# Autodesk Inventor assembly: Arm 2.0 Assembly
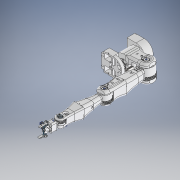
[picture p0: Inventor's stored thumbnail of the model, 180x180]
Saved by Autodesk Inventor 2017 SP1 (Build 210196100, 196)
## iProperties
Created: 2017-09-28
Part Number: Arm 2.0 Assembly
Document SubType Name: Assembly
Designer: Zach
Author: Zach
## Documents named in this file (58)
- C:\Users\Zach\Documents\GitHub\tr1\src\Body\Arm 2.0 Assembly\Arm 2.0 Assembly.iam
- C:\Users\Zach\Documents\GitHub\tr1\src\Body\Arm 2.0 Assembly\Steel Rod 8mm x 135mm.ipt
- C:\Users\Zach\Documents\GitHub\tr1\lib\22x8x8mm Bearing.ipt
- C:\Users\Zach\Documents\GitHub\tr1\src\Body\Arm 2.0 Assembly\AA004.ipt
- C:\Users\Zach\Documents\GitHub\tr1\lib\QS12MM250\QS12MM250.ipt
- C:\Users\Zach\Documents\GitHub\tr1\src\Body\Arm 2.0 Assembly\Steel Rod 8mm x 100mm.ipt
- C:\Users\Zach\Documents\GitHub\tr1\src\Body\Arm 2.0 Assembly\AA013.ipt
- C:\Users\Zach\Documents\GitHub\tr1\src\Body\Arm 2.0 Assembly\AA014.ipt
- C:\Users\Zach\Documents\GitHub\tr1\lib\12V DC Motor 378-1.ipt
- C:\Users\Zach\Documents\Inventor\Content Center Files\R2017\en-US\ISO 4017(1)\ISO 4017 - M5 x 20 - ISO.ipt
- C:\Users\Zach\Documents\GitHub\tr1\src\Body\Arm 2.0 Assembly\Steel Rod 8mm x 80mm.ipt
- C:\Users\Zach\Documents\GitHub\BCN3D-Moveo\Autodesk Inventor files\Gripper B Assembly.iam
- C:\Users\Zach\Documents\Inventor\Content Center Files\R2017\en-US\CNS 4320\CNS 4320 - M8 x 1 x 100.ipt
- C:\Users\Zach\Documents\GitHub\tr1\lib\AS 1110 - M8 x 150.ipt
- C:\Users\Zach\Documents\GitHub\tr1\lib\8mm Hub.ipt
- C:\Users\Zach\Documents\GitHub\tr1\src\Body\Arm 2.0 Assembly\Arm 2.0 Assembly\Design Accelerator\Spur Gears5.iam
- C:\Users\Zach\Documents\GitHub\tr1\lib\4mm mounting hub.ipt
- C:\Users\Zach\Documents\GitHub\tr1\lib\6201RS\6201RS.ipt
- C:\Users\Zach\Documents\GitHub\tr1\lib\U51105\U51105.ipt
- C:\Users\Zach\Documents\GitHub\tr1\src\Body\Arm 2.0 Assembly\AA031.ipt
- C:\Users\Zach\Documents\GitHub\tr1\src\Body\Arm 2.0 Assembly\AA034.ipt
- C:\Users\Zach\Documents\GitHub\tr1\src\Body\Arm 2.0 Assembly\Arm 2.0 Assembly\Design Accelerator\Spur Gears6.iam
- C:\Users\Zach\Documents\GitHub\tr1\src\Body\Arm 2.0 Assembly\AA008c.ipt
- C:\Users\Zach\Documents\GitHub\tr1\src\Body\Arm 2.0 Assembly\AA008d.ipt
- C:\Users\Zach\Documents\GitHub\tr1\src\Body\Arm 2.0 Assembly\AA035.ipt
- C:\Users\Zach\Documents\GitHub\tr1\src\Body\Arm 2.0 Assembly\Arm 2.0 Assembly\Design Accelerator\Spur Gears7.iam
- C:\Users\Zach\Documents\GitHub\tr1\src\Body\Arm 2.0 Assembly\AA036.ipt
- C:\Users\Zach\Documents\GitHub\tr1\src\Body\Arm 2.0 Assembly\AA037.ipt
- C:\Users\Zach\Documents\GitHub\tr1\src\Body\Arm 2.0 Assembly\AA016b.ipt
- C:\Users\Zach\Documents\GitHub\tr1\src\Body\Arm 2.0 Assembly\AA005b.ipt
- C:\Users\Zach\Documents\GitHub\tr1\src\Body\Arm 2.0 Assembly\AA006b.ipt
- C:\Users\Zach\Documents\GitHub\tr1\src\Body\Arm 2.0 Assembly\AA001c.ipt
- C:\Users\Zach\Documents\GitHub\tr1\lib\uxcell 12V 5RPM 8mm Worm Gear Motor\uxcell 12V 5RPM 8mm Worm Gear Motor.ipt
- C:\Users\Zach\Documents\GitHub\tr1\lib\Bourns ACE 128\Bourns ACE 128.ipt
- C:\Users\Zach\Documents\GitHub\tr1\src\Body\Arm 2.0 Assembly\Arm 2.0 Assembly\Design Accelerator\Spur Gears8.iam
- C:\Users\Zach\Documents\GitHub\tr1\src\Body\Arm 2.0 Assembly\Arm 2.0 Assembly\Design Accelerator\Spur Gears11.iam
- C:\Users\Zach\Documents\GitHub\tr1\src\Body\Arm 2.0 Assembly\Arm 2.0 Assembly\Design Accelerator\Spur Gears9.iam
- C:\Users\Zach\Documents\GitHub\tr1\src\Body\Arm 2.0 Assembly\AA010b.ipt
- C:\Users\Zach\Documents\GitHub\tr1\lib\uxcell 12V 6RPM 6mm Worm Gear Motor\uxcell 12V 6RPM 6mm Worm Gear Motor.ipt
- C:\Users\Zach\Documents\GitHub\tr1\src\Body\Arm 2.0 Assembly\Arm 2.0 Assembly\Design Accelerator\Spur Gears10.iam
- C:\Users\Zach\Documents\GitHub\tr1\src\Body\Arm 2.0 Assembly\Arm 2.0 Assembly\Design Accelerator\Spur Gears12.iam
- C:\Users\Zach\Documents\GitHub\tr1\src\Body\Arm 2.0 Assembly\AA041.ipt
- C:\Users\Zach\Documents\GitHub\tr1\src\Body\Arm 2.0 Assembly\AA042.ipt
- C:\Users\Zach\Documents\Inventor\Content Center Files\R2017\en-US\ISO 7045  H\ISO 7045 - M3 x 8 - 4.8 - H - ISO.ipt
- C:\Users\Zach\Documents\GitHub\tr1\src\Body\Arm 2.0 Assembly\AA043.ipt
- C:\Users\Zach\Documents\GitHub\tr1\src\Body\Arm 2.0 Assembly\AA044.ipt
- C:\Users\Zach\Documents\GitHub\tr1\src\Body\Arm 2.0 Assembly\AA045.ipt
- C:\Users\Zach\Documents\GitHub\tr1\src\Body\Arm 2.0 Assembly\Arm 2.0 Assembly\Design Accelerator\Spur Gears13.iam
- C:\Users\Zach\Documents\GitHub\tr1\src\Body\Arm 2.0 Assembly\Arm 2.0 Assembly\Design Accelerator\Spur Gears16.iam
- C:\Users\Zach\Documents\GitHub\tr1\src\Body\Arm 2.0 Assembly\AA046.ipt
- C:\Users\Zach\Documents\GitHub\tr1\lib\MG995.ipt
- C:\Users\Zach\Documents\GitHub\tr1\lib\Servo Mounting Hub.ipt
- C:\Users\Zach\Documents\GitHub\tr1\src\Body\Arm 2.0 Assembly\AA047.ipt
- C:\Users\Zach\Documents\GitHub\tr1\src\Body\Arm 2.0 Assembly\AA048.ipt
- C:\Users\Zach\Documents\Inventor\Content Center Files\R2017\en-US\ISO 4018\ISO 4018 - M5 x 10.ipt
- C:\Users\Zach\Documents\Inventor\Content Center Files\R2017\en-US\ISO 4018\ISO 4018 - M5 x 25.ipt
- C:\Users\Zach\Documents\Inventor\Content Center Files\R2017\en-US\ISO 7045  H\ISO 7045 - M3 x 12 - 4.8 - H - ISO.ipt
- C:\Users\Zach\Documents\GitHub\tr1\src\Body\Arm 2.0 Assembly\AA049.ipt
## Components (115 placed, 48 different names)
1. AA001c:1 — Mate:554, Mate:555, Mate:556, Mate:557, Mate:560, Flush:18, Mate:562, Mate:563, Mate:564, Mate:565, Mate:566, Mate:567, Mate:568, Mate:569, Mate:570, Mate:571, Mate:572, Mate:573, Mate:574, Mate:576, Mate:578, Mate:581, Angle:1, Mate:592, Mate:602
2. AA004:1 — Mate:23, Mate:345, Mate:347, Mate:350, Mate:357, Mate:554, Mate:555, Mate:556, Mate:590, Mate:591
3. AA005b:1 — Mate:537, Mate:538, Mate:539, Mate:541, Mate:542, Mate:543
4. AA006b:1 — Mate:544, Mate:583, Mate:584, Angle:2, Mate:588, Mate:593, Mate:594, Mate:598, Mate:599, Mate:600, Mate:609
5. AA008c:1 — Mate:449, Mate:450, Mate:451, Mate:452, Mate:453, Mate:454, Mate:463, Mate:464, Mate:466, Mate:467, Mate:481, Mate:616, Mate:662, Mate:663, Mate:751
6. AA008d:1 — Mate:455, Mate:456, Mate:457, Mate:461, Mate:463, Mate:464, Mate:466, Mate:467, Mate:614, Angle:4, Mate:635, Mate:662, Mate:663, Mate:697, Mate:699, Mate:751
7. AA010b:1 — Mate:615, Mate:616, Mate:617, Mate:618, Mate:620, Mate:621, Mate:623, Mate:624, Mate:625, Mate:626, Mate:628, Mate:630, Mate:632, Mate:633, Mate:634, Mate:636, Mate:637, Angle:6, Mate:642, Flush:20, Mate:648, Mate:650
8. AA013:2 — Mate:142, Mate:143, Mate:144, Mate:145, Mate:146, Mate:147, Mate:563, Mate:564, Mate:565
9. AA014:2 — Mate:628, Mate:629, Mate:630
10. AA016b:1 — Mate:518, Mate:519, Mate:520, Mate:521, Mate:525, Mate:526, Mate:527, Mate:529, Mate:530, Mate:664, Mate:665, Mate:667, Mate:668, Mate:669, Angle:7, Mate:671, Mate:673, Mate:675, Mate:676, Mate:677
11. AA031:1 — Mate:366, Mate:367, Mate:523, Mate:524
12. AA034:1 — Mate:529, Mate:534, Mate:535, Mate:700, Mate:701, Mate:709
13. AA035:1 — Mate:477, Mate:479, Mate:481, Mate:557, Mate:601, Mate:652, Mate:653, Mate:697, Mate:699
14. AA036:1 — Mate:498, Mate:500, Mate:501, Mate:502, Mate:511, Mate:698
15. AA037:1 — Mate:501, Mate:502, Mate:514, Mate:515, Mate:516, Mate:517, Mate:518, Mate:519, Mate:520, Mate:530, Mate:664, Mate:665, Mate:698
16. AA041:1 — Mate:675, Mate:676, Mate:677, Mate:682, Mate:683, Mate:684, Mate:685
17. AA042:1 — Mate:678, Mate:679, Mate:686, Mate:687, Angle:14
18. AA043:1 — Mate:688, Mate:689, Angle:8
19. AA043:2 — Mate:693, Mate:694, Angle:10
20. AA043:3 — Mate:742, Mate:743, Angle:13
21. AA044:1 — Mate:691, Mate:692, Angle:9
22. AA044:2 — Mate:695, Mate:696, Angle:11
23. AA045:2 — Mate:700, Mate:701, Mate:702, Mate:703, Mate:704, Mate:705, Mate:706, Mate:708, Flush:21, Mate:709, Mate:711, Mate:713, Mate:715, Mate:717, Mate:718, Angle:12, Mate:719, Mate:720, Mate:723, Mate:725, Mate:780, Mate:781, Mate:784, Mate:785
24. AA046:1 — Mate:727, Mate:728, Mate:731, Mate:735, Mate:736, Mate:737, Mate:752, Mate:756, Mate:757, Mate:758, Mate:759, Mate:760, Mate:761, Mate:762, Mate:763
25. AA047:1 — Mate:735, Mate:736, Mate:737, Mate:738, Mate:739, Mate:740, Mate:753, Mate:754, Mate:755, Mate:800, Mate:801
26. AA048:1 — Mate:744, Mate:745, Mate:746, Mate:747, Mate:748, Mate:749
27. AA049:1 — Mate:783, Mate:784, Mate:785, Mate:786, Mate:787, Mate:788, Mate:789, Mate:790, Mate:791
28. Gripper B Assembly:1 [sub-assembly] — Mate:747, Mate:748, Mate:749, Mate:750, Flush:22, Flush:23
29. 22x8x8mm Bearing:1 — Mate:433, Mate:560
30. 22x8x8mm Bearing:2 — Mate:437, Mate:562
31. 22x8x8mm Bearing:3 — Mate:57, Mate:620, Mate:626, Mate:645
32. 22x8x8mm Bearing:4 — Mate:621, Mate:629, Mate:642
33. 22x8x8mm Bearing:5 — Mate:186, Mate:708
34. 22x8x8mm Bearing:6 — Mate:187, Mate:719
35. 22x8x8mm Bearing:7 — Mate:264, Mate:526
36. 22x8x8mm Bearing:8 — Mate:527, Mate:528
37. 22x8x8mm Bearing:13 — Mate:451, Mate:452
38. 22x8x8mm Bearing:14 — Mate:449, Mate:450
39. QS12MM250:1 — Mate:23, Mate:344, Mate:346, Mate:348, Mate:354, Mate:537, Mate:544, Mate:585, Mate:593, Mate:594, Mate:597
40. Steel Rod 8mm x 135mm:1 — Mate:433, Mate:437, Mate:476, Mate:477, Flush:18, Mate:575, Mate:651
41. Steel Rod 8mm x 100mm:1 — Mate:57, Mate:491, Mate:498, Flush:20, Mate:644, Mate:649
42. Steel Rod 8mm x 80mm:1 — Mate:186, Mate:187, Mate:706, Flush:21, Mate:710, Mate:721, Mate:724, Mate:730, Mate:783
43. 12V DC Motor 378-1:3 — Mate:702, Mate:703, Mate:704, Mate:705, Mate:712, Mate:714, Mate:778, Mate:779
44. 12V DC Motor 378-1:4 — Mate:514, Mate:515, Mate:516, Mate:522
45. 12V DC Motor 378-1:6 — Mate:340, Mate:342, Mate:538, Mate:539, Mate:540, Mate:543
46. 12V DC Motor 378-1:7 — Mate:455, Mate:456, Mate:457, Mate:460, Mate:610
47. uxcell 12V 6RPM 6mm Worm Gear Motor:1 — Mate:632, Mate:633, Mate:634
48. uxcell 12V 5RPM 8mm Worm Gear Motor:1 — Mate:568, Mate:569, Mate:570, Mate:571, Mate:572
49. 6201RS:1 — Mate:346, Mate:347
50. 6201RS:2 — Mate:357, Mate:597
51. U51105:1 — Mate:348, Mate:349, Mate:542
52. U51105:2 — Mate:354, Mate:608, Mate:609
53. 8mm Hub:2 — Mate:368, Mate:531, Mate:534, Mate:535
54. 8mm Hub:3 — Mate:617, Mate:618, Mate:690
55. 8mm Hub:4 — Mate:580, Mate:581, Mate:582
56. 8mm Hub:5 — Mate:644, Mate:645, Mate:646
57. 8mm Hub:6 — Mate:651, Mate:652, Mate:653
58. 8mm Hub:7 — Mate:666, Mate:667, Mate:674
59. 8mm Hub:8 — Mate:720, Mate:721, Mate:726
60. 8mm Hub:9 — Mate:727, Mate:728, Mate:730, Mate:756, Mate:764, Mate:765, Mate:766, Mate:767, Mate:768, Mate:769
61. 4mm mounting hub:1 — Mate:340, Mate:343, Mate:540, Mate:541
62. 4mm mounting hub:3 — Mate:366, Mate:367, Mate:517, Mate:522, Mate:523, Mate:524
63. 4mm mounting hub:5 — Mate:513, Mate:622, Mate:623
64. 4mm mounting hub:7 — Mate:460, Mate:461, Mate:611, Mate:613
65. 4mm mounting hub:8 — Mate:714, Mate:715, Mate:716, Mate:782
66. Servo Mounting Hub:1 — Mate:733, Mate:734, Mate:738, Mate:739, Mate:740, Mate:792, Mate:793, Mate:794, Mate:795, Mate:796, Mate:797, Mate:798, Mate:799
67. ISO 4017 M5 x 20:1 — Mate:146, Mate:147
68. ISO 4017 M5 x 20:2 — Mate:144, Mate:145
69. ISO 4017 M5 x 20:3 — Mate:142, Mate:143
70. CNS 4320 M8 x 100:1 — Mate:264, Mate:368, Mate:521, Mate:525, Mate:528, Mate:531, Mate:666, Mate:670
71. AS 1110 - Metric M8 x 80:2 — Mate:453, Mate:454, Angle:5, Mate:615, Mate:690
72. ISO 7045 H M3 x 8 - 4.8 - H:1 — Mate:680, Mate:681
73. ISO 7045 H M3 x 8 - 4.8 - H:2 — Mate:682, Mate:685
74. ISO 7045 H M3 x 8 - 4.8 - H:3 — Mate:683, Mate:684
75. ISO 7045 H M3 x 8 - 4.8 - H:4 — Mate:686, Mate:687
76. Bourns ACE 128:1 — Mate:573, Mate:574, Mate:577, Angle:1, Mate:693, Mate:694
77. Bourns ACE 128:2 — Mate:583, Mate:584, Angle:2, Mate:587, Mate:695, Mate:696
78. Bourns ACE 128:3 — Mate:612, Mate:614, Angle:4, Mate:635, Mate:691, Mate:692
79. Bourns ACE 128:4 — Mate:636, Mate:637, Angle:6, Mate:647, Mate:688, Mate:689
80. Bourns ACE 128:5 — Mate:668, Mate:669, Angle:7, Mate:672, Mate:678, Mate:679
81. Bourns ACE 128:6 — Mate:717, Mate:718, Angle:12, Mate:722, Mate:742, Mate:743
82. Spur Gears:5 [sub-assembly] — Mate:342, Mate:343, Mate:344, Mate:345, Mate:349, Mate:350
83. Spur Gears:6 [sub-assembly] — Mate:476, Mate:479, Mate:566, Mate:567, Mate:601, Mate:602
84. Spur Gears:7 [sub-assembly] — Mate:491, Mate:500, Mate:511, Mate:513, Mate:622, Mate:624, Mate:625
85. Spur Gears:8 [sub-assembly] — Mate:575, Mate:576, Mate:577, Mate:578, Mate:580, Mate:582, Angle:10
86. Spur Gears:9 [sub-assembly] — Mate:585, Mate:587, Mate:588, Mate:590, Mate:591, Mate:592, Mate:608, Angle:11
87. Spur Gears:10 [sub-assembly] — Mate:610, Mate:611, Mate:612, Mate:613, Angle:5, Angle:9
88. Spur Gears:11 [sub-assembly] — Mate:646, Mate:647, Mate:648, Mate:649, Mate:650, Angle:8
89. Spur Gears:12 [sub-assembly] — Mate:670, Mate:671, Mate:672, Mate:673, Mate:674, Mate:680, Mate:681, Angle:14
90. Spur Gears:13 [sub-assembly] — Mate:710, Mate:711, Mate:712, Mate:713, Mate:716, Mate:731, Mate:757, Mate:770, Mate:771, Mate:772, Mate:773, Mate:774, Mate:775, Mate:776, Mate:777, Mate:782
91. Spur Gears:14 [sub-assembly] — Mate:722, Mate:723, Mate:724, Mate:725, Mate:726, Angle:13
92. MG995:1 — Mate:733, Mate:734, Mate:744, Mate:745, Mate:746
93. MG995:2 — Mate:750, Flush:22, Flush:23
94. ISO 4018 M5 x 10:1 — Mate:754, Mate:755
95. ISO 4018 M5 x 10:2 — Mate:752, Mate:753
96. ISO 4018 M5 x 25:2 — Mate:758, Mate:761
97. ISO 4018 M5 x 25:5 — Mate:759, Mate:763
98. ISO 4018 M5 x 25:6 — Mate:760, Mate:762
99. ISO 7045 H M3 x 12 - 4.8 - H:1 — Mate:765, Mate:767
100. ISO 7045 H M3 x 12 - 4.8 - H:3 — Mate:764, Mate:769
101. ISO 7045 H M3 x 12 - 4.8 - H:2 — Mate:766, Mate:768
102. ISO 7045 H M3 x 12 - 4.8 - H:4 — Mate:770, Mate:775
103. ISO 7045 H M3 x 12 - 4.8 - H:5 — Mate:771, Mate:774
104. ISO 7045 H M3 x 12 - 4.8 - H:6 — Mate:773, Mate:777
105. ISO 7045 H M3 x 12 - 4.8 - H:7 — Mate:772, Mate:776
106. ISO 7045 H M3 x 8 - 4.8 - H:5 — Mate:778, Mate:780
107. ISO 7045 H M3 x 8 - 4.8 - H:6 — Mate:779, Mate:781
108. ISO 4018 M5 x 10:5 — Mate:786, Mate:789
109. ISO 4018 M5 x 10:3 — Mate:787, Mate:790
110. ISO 4018 M5 x 10:4 — Mate:788, Mate:791
111. ISO 7045 H M3 x 8 - 4.8 - H:7 — Mate:795, Mate:799
112. ISO 7045 H M3 x 8 - 4.8 - H:8 — Mate:794, Mate:798
113. ISO 7045 H M3 x 8 - 4.8 - H:9 — Mate:792, Mate:796
114. ISO 7045 H M3 x 8 - 4.8 - H:10 — Mate:793, Mate:797
115. ISO 7045 H M3 x 8 - 4.8 - H:11 — Mate:800, Mate:801
## Relationships (315: Mate 297, Angle 13, Flush 5)
- Mate:23: AA004:1 ↔ QS12MM250:1
- Mate:57: 22x8x8mm Bearing:3 ↔ Steel Rod 8mm x 100mm:1
- Mate:142: AA013:2 ↔ ISO 4017 M5 x 20:3
- Mate:143: AA013:2 ↔ ISO 4017 M5 x 20:3
- Mate:144: AA013:2 ↔ ISO 4017 M5 x 20:2
- Mate:145: AA013:2 ↔ ISO 4017 M5 x 20:2
- Mate:146: AA013:2 ↔ ISO 4017 M5 x 20:1
- Mate:147: AA013:2 ↔ ISO 4017 M5 x 20:1
- Mate:186: 22x8x8mm Bearing:5 ↔ Steel Rod 8mm x 80mm:1
- Mate:187: 22x8x8mm Bearing:6 ↔ Steel Rod 8mm x 80mm:1
- Mate:264: 22x8x8mm Bearing:7 ↔ CNS 4320 M8 x 100:1
- Mate:340: 12V DC Motor 378-1:6 ↔ 4mm mounting hub:1
- Mate:342: 12V DC Motor 378-1:6 ↔ Spur Gears:5
- Mate:343: 4mm mounting hub:1 ↔ Spur Gears:5
- Mate:344: QS12MM250:1 ↔ Spur Gears:5
- Mate:345: AA004:1 ↔ Spur Gears:5
- Mate:346: QS12MM250:1 ↔ 6201RS:1
- Mate:347: AA004:1 ↔ 6201RS:1
- Mate:348: QS12MM250:1 ↔ U51105:1
- Mate:349: U51105:1 ↔ Spur Gears:5
- Mate:350: AA004:1 ↔ Spur Gears:5
- Mate:354: QS12MM250:1 ↔ U51105:2
- Mate:357: AA004:1 ↔ 6201RS:2
- Mate:366: AA031:1 ↔ 4mm mounting hub:3
- Mate:367: AA031:1 ↔ 4mm mounting hub:3
- Mate:368: 8mm Hub:2 ↔ CNS 4320 M8 x 100:1
- Mate:433: 22x8x8mm Bearing:1 ↔ Steel Rod 8mm x 135mm:1
- Mate:437: 22x8x8mm Bearing:2 ↔ Steel Rod 8mm x 135mm:1
- Mate:449: AA008c:1 ↔ 22x8x8mm Bearing:14
- Mate:450: AA008c:1 ↔ 22x8x8mm Bearing:14
- Mate:451: AA008c:1 ↔ 22x8x8mm Bearing:13
- Mate:452: AA008c:1 ↔ 22x8x8mm Bearing:13
- Mate:453: AA008c:1 ↔ AS 1110 - Metric M8 x 80:2
- Mate:454: AA008c:1 ↔ AS 1110 - Metric M8 x 80:2
- Mate:455: AA008d:1 ↔ 12V DC Motor 378-1:7
- Mate:456: AA008d:1 ↔ 12V DC Motor 378-1:7
- Mate:457: AA008d:1 ↔ 12V DC Motor 378-1:7
- Mate:460: 12V DC Motor 378-1:7 ↔ 4mm mounting hub:7
- Mate:461: AA008d:1 ↔ 4mm mounting hub:7
- Mate:463: AA008c:1 ↔ AA008d:1
- Mate:464: AA008c:1 ↔ AA008d:1
- Mate:466: AA008c:1 ↔ AA008d:1
- Mate:467: AA008c:1 ↔ AA008d:1
- Mate:476: Steel Rod 8mm x 135mm:1 ↔ Spur Gears:6
- Mate:477: AA035:1 ↔ Steel Rod 8mm x 135mm:1
- Mate:479: AA035:1 ↔ Spur Gears:6
- Mate:481: AA008c:1 ↔ AA035:1
- Mate:491: Steel Rod 8mm x 100mm:1 ↔ Spur Gears:7
- Mate:498: AA036:1 ↔ Steel Rod 8mm x 100mm:1
- Mate:500: AA036:1 ↔ Spur Gears:7
- Mate:501: AA036:1 ↔ AA037:1
- Mate:502: AA036:1 ↔ AA037:1
- Mate:511: AA036:1 ↔ Spur Gears:7
- Mate:513: 4mm mounting hub:5 ↔ Spur Gears:7
- Mate:514: AA037:1 ↔ 12V DC Motor 378-1:4
- Mate:515: AA037:1 ↔ 12V DC Motor 378-1:4
- Mate:516: AA037:1 ↔ 12V DC Motor 378-1:4
- Mate:517: AA037:1 ↔ 4mm mounting hub:3
- Mate:518: AA016b:1 ↔ AA037:1
- Mate:519: AA016b:1 ↔ AA037:1
- Mate:520: AA016b:1 ↔ AA037:1
- Mate:521: AA016b:1 ↔ CNS 4320 M8 x 100:1
- Mate:522: 12V DC Motor 378-1:4 ↔ 4mm mounting hub:3
- Mate:523: AA031:1 ↔ 4mm mounting hub:3
- Mate:524: AA031:1 ↔ 4mm mounting hub:3
- Mate:525: AA016b:1 ↔ CNS 4320 M8 x 100:1
- Mate:526 (0.5 mm): AA016b:1 ↔ 22x8x8mm Bearing:7
- Mate:527 (0.5 mm): AA016b:1 ↔ 22x8x8mm Bearing:8
- Mate:528: 22x8x8mm Bearing:8 ↔ CNS 4320 M8 x 100:1
- Mate:529: AA016b:1 ↔ AA034:1
- Mate:530: AA016b:1 ↔ AA037:1
- Mate:531: 8mm Hub:2 ↔ CNS 4320 M8 x 100:1
- Mate:534: AA034:1 ↔ 8mm Hub:2
- Mate:535: AA034:1 ↔ 8mm Hub:2
- Mate:537: AA005b:1 ↔ QS12MM250:1
- Mate:538: AA005b:1 ↔ 12V DC Motor 378-1:6
- Mate:539: AA005b:1 ↔ 12V DC Motor 378-1:6
- Mate:540: 12V DC Motor 378-1:6 ↔ 4mm mounting hub:1
- Mate:541: AA005b:1 ↔ 4mm mounting hub:1
- Mate:542: AA005b:1 ↔ U51105:1
- Mate:543: AA005b:1 ↔ 12V DC Motor 378-1:6
- Mate:544: AA006b:1 ↔ QS12MM250:1
- Mate:554: AA001c:1 ↔ AA004:1
- Mate:555: AA001c:1 ↔ AA004:1
- Mate:556: AA001c:1 ↔ AA004:1
- Mate:557: AA001c:1 ↔ AA035:1
- Mate:560: AA001c:1 ↔ 22x8x8mm Bearing:1
- Flush:18: AA001c:1 ↔ Steel Rod 8mm x 135mm:1
- Mate:562: AA001c:1 ↔ 22x8x8mm Bearing:2
- Mate:563: AA001c:1 ↔ AA013:2
- Mate:564: AA001c:1 ↔ AA013:2
- Mate:565: AA001c:1 ↔ AA013:2
- Mate:566: AA001c:1 ↔ Spur Gears:6
- Mate:567 (1 mm): AA001c:1 ↔ Spur Gears:6
- Mate:568: AA001c:1 ↔ uxcell 12V 5RPM 8mm Worm Gear Motor:1
- Mate:569: AA001c:1 ↔ uxcell 12V 5RPM 8mm Worm Gear Motor:1
- Mate:570: AA001c:1 ↔ uxcell 12V 5RPM 8mm Worm Gear Motor:1
- Mate:571: AA001c:1 ↔ uxcell 12V 5RPM 8mm Worm Gear Motor:1
- Mate:572: AA001c:1 ↔ uxcell 12V 5RPM 8mm Worm Gear Motor:1
- Mate:573: AA001c:1 ↔ Bourns ACE 128:1
- Mate:574: AA001c:1 ↔ Bourns ACE 128:1
- Mate:575: Steel Rod 8mm x 135mm:1 ↔ Spur Gears:8
- Mate:576: AA001c:1 ↔ Spur Gears:8
- Mate:577: Bourns ACE 128:1 ↔ Spur Gears:8
- Mate:578: AA001c:1 ↔ Spur Gears:8
- Mate:580: 8mm Hub:4 ↔ Spur Gears:8
- Mate:581: AA001c:1 ↔ 8mm Hub:4
- Mate:582: 8mm Hub:4 ↔ Spur Gears:8
- Angle:1 (0 deg): AA001c:1 ↔ Bourns ACE 128:1
- Mate:583: AA006b:1 ↔ Bourns ACE 128:2
- Mate:584: AA006b:1 ↔ Bourns ACE 128:2
- Angle:2 (0 deg): AA006b:1 ↔ Bourns ACE 128:2
- Mate:585: QS12MM250:1 ↔ Spur Gears:9
- Mate:587: Bourns ACE 128:2 ↔ Spur Gears:9
- Mate:588: AA006b:1 ↔ Spur Gears:9
- Mate:590: AA004:1 ↔ Spur Gears:9
- Mate:591: AA004:1 ↔ Spur Gears:9
- Mate:592: AA001c:1 ↔ Spur Gears:9
- Mate:593: AA006b:1 ↔ QS12MM250:1
- Mate:594: AA006b:1 ↔ QS12MM250:1
- Mate:597: QS12MM250:1 ↔ 6201RS:2
- Mate:598: AA006b:1
- Mate:599: AA006b:1
- Mate:600: AA006b:1
- Mate:601: AA035:1 ↔ Spur Gears:6
- Mate:602 (2.5 mm): AA001c:1 ↔ Spur Gears:6
- Mate:608: U51105:2 ↔ Spur Gears:9
- Mate:609: AA006b:1 ↔ U51105:2
- Mate:610: 12V DC Motor 378-1:7 ↔ Spur Gears:10
- Mate:611: 4mm mounting hub:7 ↔ Spur Gears:10
- Mate:612: Bourns ACE 128:3 ↔ Spur Gears:10
- Mate:613: 4mm mounting hub:7 ↔ Spur Gears:10
- Mate:614: AA008d:1 ↔ Bourns ACE 128:3
- Angle:4 (0 deg): AA008d:1 ↔ Bourns ACE 128:3
- Angle:5 (0 deg): AS 1110 - Metric M8 x 80:2 ↔ Spur Gears:10
- Mate:615: AA010b:1 ↔ AS 1110 - Metric M8 x 80:2
- Mate:616: AA008c:1 ↔ AA010b:1
- Mate:617: AA010b:1 ↔ 8mm Hub:3
- Mate:618: AA010b:1 ↔ 8mm Hub:3
- Mate:620: AA010b:1 ↔ 22x8x8mm Bearing:3
- Mate:621: AA010b:1 ↔ 22x8x8mm Bearing:4
- Mate:622: 4mm mounting hub:5 ↔ Spur Gears:7
- Mate:623: AA010b:1 ↔ 4mm mounting hub:5
- Mate:624: AA010b:1 ↔ Spur Gears:7
- Mate:625: AA010b:1 ↔ Spur Gears:7
- Flush:20 (0.5 mm): AA010b:1 ↔ Steel Rod 8mm x 100mm:1
- Mate:626: AA010b:1 ↔ 22x8x8mm Bearing:3
- Mate:628: AA010b:1 ↔ AA014:2
- Mate:629: AA014:2 ↔ 22x8x8mm Bearing:4
- Mate:630: AA010b:1 ↔ AA014:2
- Mate:632: AA010b:1 ↔ uxcell 12V 6RPM 6mm Worm Gear Motor:1
- Mate:633: AA010b:1 ↔ uxcell 12V 6RPM 6mm Worm Gear Motor:1
- Mate:634: AA010b:1 ↔ uxcell 12V 6RPM 6mm Worm Gear Motor:1
- Mate:635: AA008d:1 ↔ Bourns ACE 128:3
- Mate:636: AA010b:1 ↔ Bourns ACE 128:4
- Mate:637: AA010b:1 ↔ Bourns ACE 128:4
- Angle:6 (0 deg): AA010b:1 ↔ Bourns ACE 128:4
- Mate:642: AA010b:1 ↔ 22x8x8mm Bearing:4
- Mate:644: Steel Rod 8mm x 100mm:1 ↔ 8mm Hub:5
- Mate:645: 22x8x8mm Bearing:3 ↔ 8mm Hub:5
- Mate:646: 8mm Hub:5 ↔ Spur Gears:11
- Mate:647: Bourns ACE 128:4 ↔ Spur Gears:11
- Mate:648: AA010b:1 ↔ Spur Gears:11
- Mate:649: Steel Rod 8mm x 100mm:1 ↔ Spur Gears:11
- Mate:650: AA010b:1 ↔ Spur Gears:11
- Mate:651: Steel Rod 8mm x 135mm:1 ↔ 8mm Hub:6
- Mate:652: AA035:1 ↔ 8mm Hub:6
- Mate:653: AA035:1 ↔ 8mm Hub:6
- Mate:662: AA008c:1 ↔ AA008d:1
- Mate:663: AA008c:1 ↔ AA008d:1
- Mate:664: AA016b:1 ↔ AA037:1
- Mate:665: AA016b:1 ↔ AA037:1
- Mate:666: 8mm Hub:7 ↔ CNS 4320 M8 x 100:1
- Mate:667: AA016b:1 ↔ 8mm Hub:7
- Mate:668: AA016b:1 ↔ Bourns ACE 128:5
- Mate:669: AA016b:1 ↔ Bourns ACE 128:5
- Angle:7 (0 deg): AA016b:1 ↔ Bourns ACE 128:5
- Mate:670: CNS 4320 M8 x 100:1 ↔ Spur Gears:12
- Mate:671: AA016b:1 ↔ Spur Gears:12
- Mate:672: Bourns ACE 128:5 ↔ Spur Gears:12
- Mate:673: AA016b:1 ↔ Spur Gears:12
- Mate:674: 8mm Hub:7 ↔ Spur Gears:12
- Mate:675: AA016b:1 ↔ AA041:1
- Mate:676: AA016b:1 ↔ AA041:1
- Mate:677: AA016b:1 ↔ AA041:1
- Mate:678: AA042:1 ↔ Bourns ACE 128:5
- Mate:679: AA042:1 ↔ Bourns ACE 128:5
- Mate:680: ISO 7045 H M3 x 8 - 4.8 - H:1 ↔ Spur Gears:12
- Mate:681: ISO 7045 H M3 x 8 - 4.8 - H:1 ↔ Spur Gears:12
- Mate:682: AA041:1 ↔ ISO 7045 H M3 x 8 - 4.8 - H:2
- Mate:683: AA041:1 ↔ ISO 7045 H M3 x 8 - 4.8 - H:3
- Mate:684: AA041:1 ↔ ISO 7045 H M3 x 8 - 4.8 - H:3
- Mate:685: AA041:1 ↔ ISO 7045 H M3 x 8 - 4.8 - H:2
- Mate:686: AA042:1 ↔ ISO 7045 H M3 x 8 - 4.8 - H:4
- Mate:687: AA042:1 ↔ ISO 7045 H M3 x 8 - 4.8 - H:4
- Mate:688: AA043:1 ↔ Bourns ACE 128:4
- Mate:689: AA043:1 ↔ Bourns ACE 128:4
- Angle:8 (0 deg): AA043:1 ↔ Spur Gears:11
- Mate:690: 8mm Hub:3 ↔ AS 1110 - Metric M8 x 80:2
- Mate:691: AA044:1 ↔ Bourns ACE 128:3
- Mate:692: AA044:1 ↔ Bourns ACE 128:3
- Angle:9 (0 deg): AA044:1 ↔ Spur Gears:10
- Mate:693: AA043:2 ↔ Bourns ACE 128:1
- Mate:694: AA043:2 ↔ Bourns ACE 128:1
- Angle:10 (0 deg): AA043:2 ↔ Spur Gears:8
- Mate:695: AA044:2 ↔ Bourns ACE 128:2
- Mate:696: AA044:2 ↔ Bourns ACE 128:2
- Angle:11 (0 deg): AA044:2 ↔ Spur Gears:9
- Mate:697: AA008d:1 ↔ AA035:1
- Mate:698: AA036:1 ↔ AA037:1
- Mate:699: AA008d:1 ↔ AA035:1
- Mate:700: AA034:1 ↔ AA045:2
- Mate:701: AA034:1 ↔ AA045:2
- Mate:702: AA045:2 ↔ 12V DC Motor 378-1:3
- Mate:703: AA045:2 ↔ 12V DC Motor 378-1:3
- Mate:704: AA045:2 ↔ 12V DC Motor 378-1:3
- Mate:705: AA045:2 ↔ 12V DC Motor 378-1:3
- Mate:706: AA045:2 ↔ Steel Rod 8mm x 80mm:1
- Mate:708: AA045:2 ↔ 22x8x8mm Bearing:5
- Flush:21: AA045:2 ↔ Steel Rod 8mm x 80mm:1
- Mate:709: AA034:1 ↔ AA045:2
- Mate:710: Steel Rod 8mm x 80mm:1 ↔ Spur Gears:13
- Mate:711: AA045:2 ↔ Spur Gears:13
- Mate:712: 12V DC Motor 378-1:3 ↔ Spur Gears:13
- Mate:713: AA045:2 ↔ Spur Gears:13
- Mate:714: 12V DC Motor 378-1:3 ↔ 4mm mounting hub:8
- Mate:715: AA045:2 ↔ 4mm mounting hub:8
- Mate:716: 4mm mounting hub:8 ↔ Spur Gears:13
- Mate:717: AA045:2 ↔ Bourns ACE 128:6
- Mate:718: AA045:2 ↔ Bourns ACE 128:6
- Angle:12 (0 deg): AA045:2 ↔ Bourns ACE 128:6
- Mate:719: AA045:2 ↔ 22x8x8mm Bearing:6
- Mate:720: AA045:2 ↔ 8mm Hub:8
- Mate:721: Steel Rod 8mm x 80mm:1 ↔ 8mm Hub:8
- Mate:722: Bourns ACE 128:6 ↔ Spur Gears:14
- Mate:723: AA045:2 ↔ Spur Gears:14
- Mate:724: Steel Rod 8mm x 80mm:1 ↔ Spur Gears:14
- Mate:725: AA045:2 ↔ Spur Gears:14
- Mate:726: 8mm Hub:8 ↔ Spur Gears:14
- Mate:727: AA046:1 ↔ 8mm Hub:9
- Mate:728: AA046:1 ↔ 8mm Hub:9
- Mate:730: Steel Rod 8mm x 80mm:1 ↔ 8mm Hub:9
- Mate:731: AA046:1 ↔ Spur Gears:13
- Mate:733: Servo Mounting Hub:1 ↔ MG995:1
- Mate:734: Servo Mounting Hub:1 ↔ MG995:1
- Mate:735: AA046:1 ↔ AA047:1
- Mate:736: AA046:1 ↔ AA047:1
- Mate:737: AA046:1 ↔ AA047:1
- Mate:738: AA047:1 ↔ Servo Mounting Hub:1
- Mate:739: AA047:1 ↔ Servo Mounting Hub:1
- Mate:740: AA047:1 ↔ Servo Mounting Hub:1
- Mate:742: AA043:3 ↔ Bourns ACE 128:6
- Mate:743: AA043:3 ↔ Bourns ACE 128:6
- Angle:13 (0 deg): AA043:3 ↔ Spur Gears:14
- Mate:744: AA048:1 ↔ MG995:1
- Mate:745 (0.5 mm): AA048:1 ↔ MG995:1
- Mate:746 (0.5 mm): AA048:1 ↔ MG995:1
- Mate:747: AA048:1 ↔ Gripper B Assembly:1
- Mate:748: AA048:1 ↔ Gripper B Assembly:1
- Mate:749: AA048:1 ↔ Gripper B Assembly:1
- Mate:750: Gripper B Assembly:1 ↔ MG995:2
- Flush:22 (-2 mm): Gripper B Assembly:1 ↔ MG995:2
- Flush:23 (-0.5 mm): Gripper B Assembly:1 ↔ MG995:2
- Angle:14 (0 deg): AA042:1 ↔ Spur Gears:12
- Mate:751: AA008c:1 ↔ AA008d:1
- Mate:752: AA046:1 ↔ ISO 4018 M5 x 10:2
- Mate:753: AA047:1 ↔ ISO 4018 M5 x 10:2
- Mate:754: AA047:1 ↔ ISO 4018 M5 x 10:1
- Mate:755: AA047:1 ↔ ISO 4018 M5 x 10:1
- Mate:756: AA046:1 ↔ 8mm Hub:9
- Mate:757: AA046:1 ↔ Spur Gears:13
- Mate:758: AA046:1 ↔ ISO 4018 M5 x 25:2
- Mate:759: AA046:1 ↔ ISO 4018 M5 x 25:5
- Mate:760: AA046:1 ↔ ISO 4018 M5 x 25:6
- Mate:761: AA046:1 ↔ ISO 4018 M5 x 25:2
- Mate:762: AA046:1 ↔ ISO 4018 M5 x 25:6
- Mate:763: AA046:1 ↔ ISO 4018 M5 x 25:5
- Mate:764: 8mm Hub:9 ↔ ISO 7045 H M3 x 12 - 4.8 - H:3
- Mate:765: 8mm Hub:9 ↔ ISO 7045 H M3 x 12 - 4.8 - H:1
- Mate:766: 8mm Hub:9 ↔ ISO 7045 H M3 x 12 - 4.8 - H:2
- Mate:767: 8mm Hub:9 ↔ ISO 7045 H M3 x 12 - 4.8 - H:1
- Mate:768: 8mm Hub:9 ↔ ISO 7045 H M3 x 12 - 4.8 - H:2
- Mate:769: 8mm Hub:9 ↔ ISO 7045 H M3 x 12 - 4.8 - H:3
- Mate:770: Spur Gears:13 ↔ ISO 7045 H M3 x 12 - 4.8 - H:4
- Mate:771: Spur Gears:13 ↔ ISO 7045 H M3 x 12 - 4.8 - H:5
- Mate:772: Spur Gears:13 ↔ ISO 7045 H M3 x 12 - 4.8 - H:7
- Mate:773: Spur Gears:13 ↔ ISO 7045 H M3 x 12 - 4.8 - H:6
- Mate:774: Spur Gears:13 ↔ ISO 7045 H M3 x 12 - 4.8 - H:5
- Mate:775: Spur Gears:13 ↔ ISO 7045 H M3 x 12 - 4.8 - H:4
- Mate:776: Spur Gears:13 ↔ ISO 7045 H M3 x 12 - 4.8 - H:7
- Mate:777: Spur Gears:13 ↔ ISO 7045 H M3 x 12 - 4.8 - H:6
- Mate:778: 12V DC Motor 378-1:3 ↔ ISO 7045 H M3 x 8 - 4.8 - H:5
- Mate:779: 12V DC Motor 378-1:3 ↔ ISO 7045 H M3 x 8 - 4.8 - H:6
- Mate:780: AA045:2 ↔ ISO 7045 H M3 x 8 - 4.8 - H:5
- Mate:781: AA045:2 ↔ ISO 7045 H M3 x 8 - 4.8 - H:6
- Mate:782: 4mm mounting hub:8 ↔ Spur Gears:13
- Mate:783: AA049:1 ↔ Steel Rod 8mm x 80mm:1
- Mate:784: AA045:2 ↔ AA049:1
- Mate:785: AA045:2 ↔ AA049:1
- Mate:786: AA049:1 ↔ ISO 4018 M5 x 10:5
- Mate:787: AA049:1 ↔ ISO 4018 M5 x 10:3
- Mate:788: AA049:1 ↔ ISO 4018 M5 x 10:4
- Mate:789: AA049:1 ↔ ISO 4018 M5 x 10:5
- Mate:790: AA049:1 ↔ ISO 4018 M5 x 10:3
- Mate:791: AA049:1 ↔ ISO 4018 M5 x 10:4
- Mate:792: Servo Mounting Hub:1 ↔ ISO 7045 H M3 x 8 - 4.8 - H:9
- Mate:793: Servo Mounting Hub:1 ↔ ISO 7045 H M3 x 8 - 4.8 - H:10
- Mate:794: Servo Mounting Hub:1 ↔ ISO 7045 H M3 x 8 - 4.8 - H:8
- Mate:795: Servo Mounting Hub:1 ↔ ISO 7045 H M3 x 8 - 4.8 - H:7
- Mate:796: Servo Mounting Hub:1 ↔ ISO 7045 H M3 x 8 - 4.8 - H:9
- Mate:797: Servo Mounting Hub:1 ↔ ISO 7045 H M3 x 8 - 4.8 - H:10
- Mate:798: Servo Mounting Hub:1 ↔ ISO 7045 H M3 x 8 - 4.8 - H:8
- Mate:799: Servo Mounting Hub:1 ↔ ISO 7045 H M3 x 8 - 4.8 - H:7
- Mate:800: AA047:1 ↔ ISO 7045 H M3 x 8 - 4.8 - H:11
- Mate:801: AA047:1 ↔ ISO 7045 H M3 x 8 - 4.8 - H:11
